# Autodesk Inventor assembly: BatteryInMount
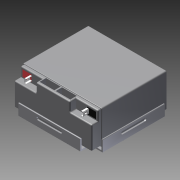
[picture p0: Inventor's stored thumbnail of the model, 180x180]
Saved by Autodesk Inventor 2012 (Build 160160000, 160)
## iProperties
Created: 2012-01-10
Part Number: BatteryInMount
Document SubType Name: Assembly
Designer: William
Author: William
## Documents named in this file (3)
- C:\Users\William\Dropbox\Robotics\CAD\team1885frc\Robot2012\Concepts\Electronics Board\BatteryInMount.iam
- C:\Users\William\Dropbox\Robotics\CAD\team1885frc\Electronics\Battery.ipt
- C:\Users\William\Dropbox\Robotics\CAD\team1885frc\Robot2012\Concepts\Electronics Board\BatteryMountSide.ipt
## Components (5 placed, 2 different names)
1. Battery:1 — Mate:1, Mate:2, Mate:3, Mate:4, Mate:5, Mate:6, Mate:7, Mate:8, Mate:11, Mate:12
2. BatteryMountSide:1 — Mate:1, Mate:5, Mate:11
3. BatteryMountSide:2 — Mate:2, Mate:6, Mate:9
4. BatteryMountSide:3 — Mate:3, Mate:7, Mate:10
5. BatteryMountSide:4 — Mate:4, Mate:8, Mate:9, Mate:10, Mate:12
## Relationships (12: Mate 12)
- Mate:1: Battery:1 ↔ BatteryMountSide:1
- Mate:2: Battery:1 ↔ BatteryMountSide:2
- Mate:3: Battery:1 ↔ BatteryMountSide:3
- Mate:4: Battery:1 ↔ BatteryMountSide:4
- Mate:5 (5.08 mm): Battery:1 ↔ BatteryMountSide:1
- Mate:6 (5.08 mm): Battery:1 ↔ BatteryMountSide:2
- Mate:7 (5.08 mm): Battery:1 ↔ BatteryMountSide:3
- Mate:8 (5.08 mm): Battery:1 ↔ BatteryMountSide:4
- Mate:9 (1.905 mm): BatteryMountSide:2 ↔ BatteryMountSide:4
- Mate:10 (1.905 mm): BatteryMountSide:3 ↔ BatteryMountSide:4
- Mate:11 (12.446 mm): Battery:1 ↔ BatteryMountSide:1
- Mate:12 (12.446 mm): Battery:1 ↔ BatteryMountSide:4
